# Autodesk Inventor assembly: robot
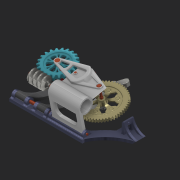
[picture p0: Inventor's stored thumbnail of the model, 180x180]
Saved by Autodesk Inventor 2020 (Build 240168000, 168)
## iProperties
Created: 2020-07-14
Part Number: robot
Document SubType Name: Assembly
Designer: alons
Author: alons
## Documents named in this file (18)
- C:\Users\alons\OneDrive\Documents\GitHub\Water-Strider-Robot\Striderbot\robot.iam
- C:\Users\alons\OneDrive\Documents\GitHub\Water-Strider-Robot\Striderbot\spur_gears_mesh_2\Design Accelerator\Spur Gear13.ipt
- C:\Users\alons\OneDrive\Documents\GitHub\Water-Strider-Robot\Striderbot\spur_gears_mesh_2\Design Accelerator\Spur Gear23.ipt
- C:\Users\alons\OneDrive\Documents\GitHub\Water-Strider-Robot\Striderbot\spur_gears_mesh_3\Design Accelerator\Spur Gear11.ipt
- C:\Users\alons\OneDrive\Documents\GitHub\Water-Strider-Robot\Striderbot\spur_gears_mesh_3\Design Accelerator\Spur Gear21.ipt
- C:\Users\alons\OneDrive\Documents\GitHub\Water-Strider-Robot\Striderbot\worm_gear_mesh_1\Design Accelerator\Worm Gear14.ipt
- C:\Users\alons\OneDrive\Documents\GitHub\Water-Strider-Robot\Striderbot\Crank_Rocker\Link_1.ipt
- C:\Users\alons\OneDrive\Documents\GitHub\Water-Strider-Robot\Striderbot\Crank_Rocker\Link_2.ipt
- C:\Users\alons\OneDrive\Documents\GitHub\Water-Strider-Robot\Striderbot\Crank_Rocker\Link_3.ipt
- C:\Users\alons\OneDrive\Documents\GitHub\Water-Strider-Robot\Striderbot\worm_gear_mesh_1\Design Accelerator\Worm14.ipt
- C:\Users\alons\OneDrive\Documents\GitHub\Water-Strider-Robot\Striderbot\Machine_Frame\top_frame.ipt
- C:\Users\alons\OneDrive\Documents\GitHub\Water-Strider-Robot\Striderbot\Machine_Frame\bottom_frame.ipt
- C:\Users\alons\OneDrive\Documents\GitHub\Water-Strider-Robot\Striderbot\Machine_Frame\bottom_frame_2.ipt
- C:\Users\alons\OneDrive\Documents\GitHub\Water-Strider-Robot\Striderbot\Shaft1.ipt
- C:\Users\alons\OneDrive\Documents\GitHub\Water-Strider-Robot\Striderbot\Shaft2.ipt
- C:\Users\alons\OneDrive\Documents\GitHub\Water-Strider-Robot\Striderbot\Shaft5.ipt
- C:\Users\alons\OneDrive\Documents\GitHub\Water-Strider-Robot\Striderbot\Shaft3.ipt
- C:\Users\alons\OneDrive\Documents\GitHub\Water-Strider-Robot\Striderbot\Shaft4.ipt
## Components (17 placed, 13 different names)
1. Spur Gear1:1 — Flush:1, Mate:3, Rotation:1, Mate:10, Mate:11, Mate:34, Mate:43
2. Spur Gear2:1 — Flush:1, Mate:3, Rotation:1, Flush:2, Mate:6, Mate:39, Mate:56
3. Spur Gear1:2 — Flush:2, Mate:6, Flush:3, Mate:7, Rotation:3, Mate:19, Mate:35
4. Spur Gear2:2 — Flush:3, Mate:7, Rotation:3, Mate:12, Mate:13, Mate:14, Flush:7, Mate:40
5. Worm Gear:1 — Mate:10, Mate:11, Rotation:4, Mate:32, Mate:42
6. Link_1:1 — Mate:12, Mate:13, Mate:14, Mate:15, Mate:16
7. Link_2:1 — Mate:15, Mate:16, Mate:17, Mate:18
8. Link_3:1 — Mate:17, Mate:18, Mate:19, Mate:44
9. Worm:1 — Rotation:4, Mate:33, Mate:38, Flush:8, Mate:53
10. top_frame:1 — Mate:25, Mate:26, Mate:32, Mate:33, Mate:34, Mate:35, Mate:38, Flush:8, Mate:39, Mate:40, Mate:42, Mate:45, Mate:48, Mate:49, Mate:52, Mate:54, Mate:55, Mate:57
11. bottom_frame:1 — Mate:25, Mate:26, Mate:41, Mate:46, Mate:47, Flush:9, Mate:50, Mate:51
12. bottom_frame_2:1 — Mate:43, Mate:44, Mate:45
13. Driving_Shaft — Mate:48, Mate:49
14. Frame_Shaft — Mate:50, Mate:51
15. Shaft:2 — Mate:54, Mate:55
16. Shaft:3 — Mate:56, Mate:57
17. Shaft:4 — Mate:52, Mate:53
## Relationships (48: Mate 39, Flush 6, RelateRotation 3)
- Flush:1: Spur Gear1:1 ↔ Spur Gear2:1
- Mate:3 (6.3 mm): Spur Gear1:1 ↔ Spur Gear2:1
- Rotation:1 [RelateRotation] (0.7812 ul): Spur Gear1:1 ↔ Spur Gear2:1
- Flush:2: Spur Gear2:1 ↔ Spur Gear1:2
- Mate:6: Spur Gear2:1 ↔ Spur Gear1:2
- Flush:3: Spur Gear1:2 ↔ Spur Gear2:2
- Mate:7 (8.45 mm): Spur Gear1:2 ↔ Spur Gear2:2
- Rotation:3 [RelateRotation] (0.789 ul): Spur Gear1:2 ↔ Spur Gear2:2
- Mate:10: Spur Gear1:1 ↔ Worm Gear:1
- Mate:11: Spur Gear1:1 ↔ Worm Gear:1
- Mate:12: Spur Gear2:2 ↔ Link_1:1
- Mate:13: Spur Gear2:2 ↔ Link_1:1
- Mate:14 (1.3 mm): Spur Gear2:2 ↔ Link_1:1
- Mate:15: Link_1:1 ↔ Link_2:1
- Mate:16: Link_1:1 ↔ Link_2:1
- Mate:17: Link_2:1 ↔ Link_3:1
- Mate:18: Link_2:1 ↔ Link_3:1
- Mate:19: Spur Gear1:2 ↔ Link_3:1
- Rotation:4 [RelateRotation] (0.0455 ul): Worm Gear:1 ↔ Worm:1
- Mate:25: top_frame:1 ↔ bottom_frame:1
- Flush:7: Spur Gear2:2
- Mate:26: top_frame:1 ↔ bottom_frame:1
- Mate:32: Worm Gear:1 ↔ top_frame:1
- Mate:33: Worm:1 ↔ top_frame:1
- Mate:34 (-2 mm): Spur Gear1:1 ↔ top_frame:1
- Mate:35 (-4.2 mm): Spur Gear1:2 ↔ top_frame:1
- Mate:38: Worm:1 ↔ top_frame:1
- Flush:8 (13.55 mm): Worm:1 ↔ top_frame:1
- Mate:39 (-6.8 mm): Spur Gear2:1 ↔ top_frame:1
- Mate:40 (-6.8 mm): Spur Gear2:2 ↔ top_frame:1
- Mate:41: bottom_frame:1
- Mate:42: Worm Gear:1 ↔ top_frame:1
- Mate:43: Spur Gear1:1 ↔ bottom_frame_2:1
- Mate:44: Link_3:1 ↔ bottom_frame_2:1
- Mate:45: top_frame:1 ↔ bottom_frame_2:1
- Mate:46: bottom_frame:1
- Mate:47: bottom_frame:1
- Flush:9: bottom_frame:1
- Mate:48: top_frame:1 ↔ Driving_Shaft
- Mate:49: top_frame:1 ↔ Driving_Shaft
- Mate:50: bottom_frame:1 ↔ Frame_Shaft
- Mate:51: bottom_frame:1 ↔ Frame_Shaft
- Mate:52: top_frame:1 ↔ Shaft:4
- Mate:53: Worm:1 ↔ Shaft:4
- Mate:54: top_frame:1 ↔ Shaft:2
- Mate:55: top_frame:1 ↔ Shaft:2
- Mate:56: Spur Gear2:1 ↔ Shaft:3
- Mate:57: top_frame:1 ↔ Shaft:3
